# Autodesk Inventor assembly: Assembly3
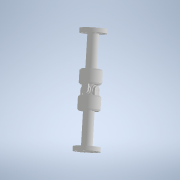
[picture p0: Inventor's stored thumbnail of the model, 180x180]
Saved by Autodesk Inventor 2021 (Build 250183000, 183)
## iProperties
Created: 2021-05-13
Part Number: Assembly3
Document SubType Name: Assembly
Designer: peris
Author: peris
## Documents named in this file (7)
- D:\Inventor\nm20003_Assembly3.iam
- D:\Inventor\nm20003_Part3.1.ipt
- D:\Inventor\nm20003_Part3.4.ipt
- D:\Inventor\nm20003_Part3.3.ipt
- D:\Inventor\nm20003_Part3.2.ipt
- D:\Inventor\nm20003_Part3.4_MIR.ipt
- D:\Inventor\nm20003_Part3.3_MIR.ipt
## Components (7 placed, 6 different names)
1. nm20003_Part3.1:1 — Mate:8
2. nm20003_Part3.4:1
3. nm20003_Part3.3:1 — Mate:8
4. nm20003_Part3.2:1
5. nm20003_Part3.1:2
6. nm20003_Part3.4_MIR:1
7. nm20003_Part3.3_MIR:1
## Relationships (18: Mate 8, Tangent 6, Flush 2, CylindricalJoint 1, Angle 1)
- [CylindricalJoint]: nm20003_Part3.1:1 ↔ nm20003_Part3.4:1
- [Mate]: nm20003_Part3.4:1 ↔ nm20003_Part3.3:1
- [Mate]: nm20003_Part3.4:1 ↔ nm20003_Part3.3:1
- [Tangent]: nm20003_Part3.4:1 ↔ nm20003_Part3.3:1
- [Mate]: nm20003_Part3.1:1 ↔ nm20003_Part3.4:1
- [Tangent]: nm20003_Part3.1:1 ↔ nm20003_Part3.3:1
- [Flush]: nm20003_Part3.1:1 ↔ nm20003_Part3.2:1
- [Tangent]: nm20003_Part3.1:1 ↔ nm20003_Part3.2:1
- [Flush]: nm20003_Part3.2:1 ↔ nm20003_Part3.1:2
- [Tangent]: nm20003_Part3.2:1 ↔ nm20003_Part3.1:2
- [Angle] (0 deg): nm20003_Part3.1:1 ↔ nm20003_Part3.1:2
- [Tangent]: nm20003_Part3.4_MIR:1 ↔ nm20003_Part3.3_MIR:1
- [Mate]: nm20003_Part3.4_MIR:1 ↔ nm20003_Part3.3_MIR:1
- [Mate]: nm20003_Part3.4_MIR:1 ↔ nm20003_Part3.3_MIR:1
- [Mate]: nm20003_Part3.1:2 ↔ nm20003_Part3.3_MIR:1
- [Mate]: nm20003_Part3.1:2 ↔ nm20003_Part3.3_MIR:1
- [Tangent]: nm20003_Part3.1:2 ↔ nm20003_Part3.3_MIR:1
- Mate:8: nm20003_Part3.1:1 ↔ nm20003_Part3.3:1
## Named parameters: d0_d2 = 0 mm, d1_d3 = 0 mm, d2_d4 = 0 mm, d3_d5 = 0 mm, d4_d6 = 0 mm, d5_d17 = 0 mm
